# Autodesk Inventor assembly: PruebaIntegracion
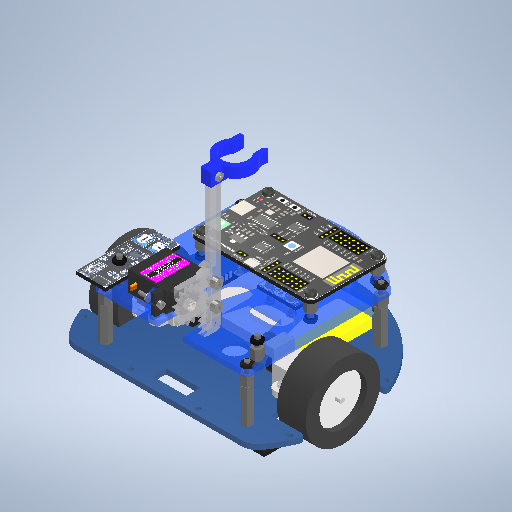
[picture p0: Inventor's stored thumbnail of the model, 512x512]
Saved by Autodesk Inventor 2025.2 (Build 292293000, 293)
## iProperties
Created: 2025-04-23
Part Number: PruebaIntegracion
Document SubType Name: Assembly
Designer: cdavi
Author: cdavi
## Documents named in this file (34)
- D:\Documentos\GIRoM\Atta-Bot-STEM\Chasis\Rediseño_Diego&Carlos\PruebaIntegracion.iam
- D:\Documentos\GIRoM\Atta-Bot-STEM\Chasis\Rediseño_Diego&Carlos\base_chasis_v5\base_chasis_v4-dimsAjustadas.ipt
- D:\Documentos\GIRoM\Atta-Bot-STEM\Chasis\Rediseño_Diego&Carlos\base_chasis_v5.ipt
- D:\Documentos\GIRoM\Atta-Bot-STEM\Chasis\Rediseño_Diego&Carlos\base_nivel2.ipt
- D:\Documentos\GIRoM\Atta-Bot-STEM\Chasis\Rediseño_Diego&Carlos\spacers\hexagonal_spacer_MF_M3_H20_HEX5.5_FTD6_MTL6.ipt
- D:\Documentos\GIRoM\Atta-Bot-STEM\Chasis\Rediseño_Diego&Carlos\spacers\hexagonal_spacer_MF_M3_H06_HEX5.5_FTD3_MTL6.ipt
- D:\Documentos\GIRoM\Atta-Bot-STEM\Chasis\Rediseño_Diego&Carlos\base_powerboost.ipt
- D:\Documentos\GIRoM\Atta-Bot-STEM\Chasis\Rediseño_Diego&Carlos\ideaboard.ipt
- D:\Documentos\Inventor\Content Center Files\R2025\en-US\ISO 4032(2)\ISO 4032 - M3 - ISO.ipt
- D:\Documentos\GIRoM\Atta-Bot-STEM\Chasis\Rediseño_Diego&Carlos\sensorFrontal.ipt
- D:\Documentos\Inventor\Content Center Files\R2025\en-US\ISO 7045  Z\ISO 7045 - M3 x 6_ - 4.8 - Z - ISO.ipt
- D:\Documentos\GIRoM\Atta-Bot-STEM\Chasis\Rediseño_Diego&Carlos\sensorInferior.ipt
- D:\Documentos\GIRoM\Atta-Bot-STEM\Chasis\Rediseño_Diego&Carlos\powerboost.ipt
- D:\Documentos\Inventor\Content Center Files\R2025\en-US\ISO 4762(2)\ISO 4762 - M2 x 8ISO.ipt
- D:\Documentos\Inventor\Content Center Files\R2025\en-US\ISO 4032(2)\ISO 4032 - M2 - ISO.ipt
- D:\Documentos\GIRoM\Atta-Bot-STEM\Chasis\Rediseño_Diego&Carlos\bateria.ipt
- D:\Documentos\GIRoM\Atta-Bot-STEM\Chasis\Rediseño_Diego&Carlos\soporteMotor.ipt
- D:\Documentos\GIRoM\Atta-Bot-STEM\Chasis\Rediseño_Diego&Carlos\motor.ipt
- D:\Documentos\GIRoM\Atta-Bot-STEM\Chasis\Rediseño_Diego&Carlos\llanta.ipt
- D:\Documentos\GIRoM\Atta-Bot-STEM\Chasis\Rediseño_Diego&Carlos\ball_caster.ipt
- D:\Documentos\Inventor\Content Center Files\R2025\en-US\ISO 4762(2)\ISO 4762 - M2 x 12ISO.ipt
- D:\Documentos\GIRoM\Atta-Bot-STEM\Chasis\Rediseño_Diego&Carlos\switch.ipt
- D:\Documentos\GIRoM\Atta-Bot-STEM\Chasis\Rediseño_Diego&Carlos\Tower Pro MG90S Micro servo.ipt
- D:\Documentos\GIRoM\Atta-Bot-STEM\Chasis\Rediseño_Diego&Carlos\EngraneMod_v2.ipt
- D:\Documentos\GIRoM\Atta-Bot-STEM\Chasis\Rediseño_Diego&Carlos\sujetador_cremallera.ipt
- D:\Documentos\GIRoM\Atta-Bot-STEM\Chasis\Rediseño_Diego&Carlos\cremallera_v2\cremallera-01.ipt
- D:\Documentos\GIRoM\Atta-Bot-STEM\Chasis\Rediseño_Diego&Carlos\cremallera_v2.ipt
- D:\Documentos\GIRoM\Atta-Bot-STEM\Chasis\Rediseño_Diego&Carlos\sujetador_marcador_v2.ipt
- D:\Documentos\Inventor\Content Center Files\R2025\en-US\ISO 7045  Z\ISO 7045 - M1,6 x 6_ - 4.8 - Z - ISO.ipt
- D:\Documentos\Inventor\Content Center Files\R2025\en-US\ISO 4762(2)\ISO 4762 - M3 x 8ISO.ipt
- D:\Documentos\GIRoM\Atta-Bot-STEM\Chasis\Rediseño_Diego&Carlos\SoporteServo.ipt
- D:\Documentos\2025\Semestre 1\Robótica\Proyecto\carcasa_v2.4.ipt
- D:\Documentos\GIRoM\Atta-Bot-STEM\Chasis\Rediseño_Diego&Carlos\spacers\hexagonal_spacer_MF_M3_H08_HEX5_FTD4_MTL8.ipt
- D:\Documentos\Inventor\Content Center Files\R2025\en-US\ISO 4762(2)\ISO 4762 - M3 x 12ISO.ipt
## Components (110 placed, 31 different names)
1. carcasa_v2.4:1 — Mate:183, Mate:184, Mate:185
2. hexagonal_spacer_MF_M3_H20_HEX5.5_FTD6_MTL6:1 — Mate:3, Mate:4
3. hexagonal_spacer_MF_M3_H20_HEX5.5_FTD6_MTL6:2 — Mate:5, Mate:6
4. hexagonal_spacer_MF_M3_H20_HEX5.5_FTD6_MTL6:3 — Mate:7, Mate:8
5. hexagonal_spacer_MF_M3_H20_HEX5.5_FTD6_MTL6:4 — Mate:9, Mate:10
6. hexagonal_spacer_MF_M3_H06_HEX5.5_FTD3_MTL6:7
7. hexagonal_spacer_MF_M3_H06_HEX5.5_FTD3_MTL6:8
8. hexagonal_spacer_MF_M3_H06_HEX5.5_FTD3_MTL6:9
9. hexagonal_spacer_MF_M3_H06_HEX5.5_FTD3_MTL6:10
10. hexagonal_spacer_MF_M3_H08_HEX5_FTD4_MTL8:2
11. hexagonal_spacer_MF_M3_H08_HEX5_FTD4_MTL8:1
12. hexagonal_spacer_MF_M3_H08_HEX5_FTD4_MTL8:3
13. hexagonal_spacer_MF_M3_H08_HEX5_FTD4_MTL8:4
14. hexagonal_spacer_MF_M3_H06_HEX5.5_FTD3_MTL6:2 — Mate:44, Mate:45
15. hexagonal_spacer_MF_M3_H06_HEX5.5_FTD3_MTL6:3 — Mate:48, Mate:49
16. hexagonal_spacer_MF_M3_H06_HEX5.5_FTD3_MTL6:1 — Mate:42, Mate:43, Mate:50, Mate:51
17. hexagonal_spacer_MF_M3_H06_HEX5.5_FTD3_MTL6:4 — Mate:46, Mate:47, Mate:52
18. hexagonal_spacer_MF_M3_H06_HEX5.5_FTD3_MTL6:5 — Mate:53, Mate:54, Mate:68, Mate:69, Mate:70
19. hexagonal_spacer_MF_M3_H06_HEX5.5_FTD3_MTL6:6 — Mate:55, Mate:56, Mate:66, Mate:67, Mate:73
20. ISO 4032 M3:17 — Mate:199, Mate:83
21. ISO 4032 M3:18 — Mate:201, Mate:85
22. ISO 7045 Z M3 x 6 - 4.8 - Z:11 — Insert:14
23. ISO 7045 Z M3 x 6 - 4.8 - Z:12 — Insert:15
24. ISO 4032 M3:13 — Insert:16
25. ISO 4032 M3:14 — Insert:17
26. ISO 4032 M3:15 — Insert:18
27. ISO 4032 M3:16 — Insert:19
28. ISO 4032 M3:7 — Insert:5
29. ISO 4032 M3:8 — Insert:6
30. ISO 4032 M3:9 — Insert:7
31. ISO 4032 M3:10 — Insert:8
32. ISO 7045 Z M3 x 6 - 4.8 - Z:10 — Insert:9
33. ISO 7045 Z M3 x 6 - 4.8 - Z:9 — Insert:10
34. ISO 4762 M3 x 12:1 — Insert:114
35. ISO 4762 M3 x 12:2 — Mate:115, Mate:116
36. ISO 7045 Z M3 x 6 - 4.8 - Z:5 — Mate:89, Mate:90
37. ISO 7045 Z M3 x 6 - 4.8 - Z:6 — Mate:91, Mate:92
38. ISO 7045 Z M3 x 6 - 4.8 - Z:7 — Mate:93, Mate:94
39. ISO 7045 Z M3 x 6 - 4.8 - Z:8 — Mate:95, Mate:96
40. ISO 4032 M3:1 — Mate:58
41. ISO 4032 M3:2 — Mate:60
42. ISO 4032 M3:3 — Mate:63
43. ISO 4032 M3:4 — Mate:64
44. ISO 4032 M3:5 — Mate:70, Mate:71
45. ISO 4032 M3:6 — Mate:72, Mate:73
46. ISO 7045 Z M3 x 6 - 4.8 - Z:1 — Mate:74, Mate:75
47. ISO 7045 Z M3 x 6 - 4.8 - Z:2 — Mate:76, Mate:77
48. ISO 7045 Z M3 x 6 - 4.8 - Z:3 — Mate:78, Mate:79
49. ISO 7045 Z M3 x 6 - 4.8 - Z:4 — Mate:80, Mate:81
50. ISO 4032 M2:14 — Mate:189, Mate:190
51. ISO 4032 M2:15 — Mate:191, Mate:192
52. ISO 4032 M2:16 — Mate:193, Mate:194, Mate:197
53. ISO 4032 M2:17 — Mate:195, Mate:196
54. ISO 4762 M2 x 8:4 — Mate:148, Mate:149, Mate:154
55. ISO 4762 M2 x 8:5 — Mate:150, Mate:151, Mate:152
56. ISO 4032 M2:6 — Mate:152, Mate:153
57. ISO 4032 M2:7 — Mate:154, Mate:155
58. ISO 4032 M2:8 — Mate:160, Mate:161
59. ISO 4032 M2:9 — Mate:162, Mate:163
60. ISO 4032 M2:10 — Mate:164, Mate:165
61. ISO 4032 M2:11 — Mate:166, Mate:167
62. ISO 4762 M2 x 8:9 — Mate:160
63. ISO 4762 M2 x 8:6 — Mate:162
64. ISO 4762 M2 x 8:7 — Mate:166
65. ISO 4762 M2 x 8:8 — Mate:164
66. ISO 4762 M2 x 8:1 — Mate:97, Mate:98, Mate:110, Mate:191
67. ISO 4762 M2 x 8:2 — Mate:99, Mate:100, Mate:112, Mate:189
68. ISO 4762 M2 x 12:2 — Mate:101, Mate:102, Mate:105, Mate:195
69. ISO 4762 M2 x 12:3 — Mate:103, Mate:104, Mate:108, Mate:193
70. ISO 4032 M2:1 — Mate:105, Mate:106
71. ISO 4032 M2:2 — Mate:107, Mate:108
72. ISO 4032 M2:3 — Mate:109, Mate:110
73. ISO 4032 M2:4 — Mate:111, Mate:112
74. ISO 7045 Z M1,6 x 6 - 4.8 - Z:2 — Mate:156, Mate:157
75. ISO 7045 Z M1,6 x 6 - 4.8 - Z:1 — Mate:158, Mate:159
76. bateria:1 — Mate:119, Mate:120
77. soporteMotor:1 — Mate:117, Mate:118, Angle:8, Mate:124, Tangent:2
78. soporteMotor:2 — Mate:119, Mate:122, Tangent:1, Mate:181, Angle:12, Mate:182
79. motor:1 — Mate:122, Tangent:1, Mate:123, Mate:126, Flush:5, Mate:127
80. motor:2 — Mate:124, Tangent:2, Mate:125, Mate:128, Mate:129, Flush:6
81. llanta:1 — Mate:126, Flush:5, Mate:127
82. llanta:2 — Mate:128, Mate:129, Flush:6
83. ball_caster:1 — Tangent:3, Tangent:7, Mate:130, Mate:156, Mate:158
84. switch:1 — Mate:131, Mate:132, Mate:133, Mate:148, Mate:149, Mate:150, Mate:151
85. sensorInferior:2 — Angle:7, Mate:85, Insert:114, Mate:82
86. sensorInferior:1 — Angle:6, Mate:83, Mate:115, Mate:116, Mate:84
87. powerboost:1 — Mate:86, Mate:87, Mate:88, Mate:97, Mate:98, Mate:99, Mate:100, Mate:101, Mate:102, Mate:103, Mate:104, Mate:197
88. base_chasis_v4-dimsAjustadas:1 — Mate:1, Flush:8, Flush:4, Mate:3, Mate:4, Mate:5, Mate:6, Mate:7, Mate:8, Mate:9, Mate:10, Mate:82, Angle:6, Mate:84, Angle:7, Mate:117, Mate:118, Angle:8, Mate:120, Mate:123, Mate:125, Tangent:3, Tangent:7, Mate:130, Mate:131, Mate:132, Mate:133, Mate:153, Mate:155, Mate:157, Mate:159, Mate:161, Mate:163, Mate:165, Mate:167, Insert:5, Insert:6, Insert:7, Insert:8, Insert:9, Insert:10, Mate:181, Angle:12, Mate:182, Mate:183, Mate:184, Mate:185, Mate:199, Mate:201
89. base_powerboost:1 — Mate:86, Mate:87, Mate:88, Mate:89, Mate:90, Mate:91, Mate:92, Mate:93, Mate:94, Mate:95, Mate:96, Mate:106, Mate:107, Mate:109, Mate:111, Mate:190, Mate:192, Mate:194, Mate:196
90. SoporteServo:2 — Mate:186, Mate:187, Mate:188, Mate:209
91. base_nivel2:1 — Mate:42, Mate:43, Mate:44, Mate:45, Mate:46, Mate:47, Mate:48, Mate:49, Mate:53, Mate:54, Mate:55, Mate:56, Mate:58, Mate:60, Mate:63, Mate:64, Angle:4, Angle:5, Angle:9, Insert:14, Insert:15, Insert:16, Insert:17, Insert:18, Insert:19, Flush:7, Mate:186, Mate:187
92. SoporteServo:1 — Mate:208
93. ideaboard:1 — Mate:50, Mate:51, Mate:52, Mate:74, Mate:75, Mate:76, Mate:77, Mate:78, Mate:79, Mate:80, Mate:81
94. sensorFrontal:1 — Mate:66, Mate:67, Angle:4, Mate:72
95. sensorFrontal:2 — Mate:68, Mate:69, Angle:5, Mate:71
96. ISO 4032 M2:13 — Mate:179, Mate:208
97. ISO 4032 M2:12 — Mate:177, Mate:209
98. ISO 4762 M2 x 12:5 — Insert:13, Mate:177
99. ISO 4762 M3 x 8:1 — Mate:202, Mate:203, Mate:206
100. ISO 4762 M3 x 8:2 — Mate:204, Mate:205, Mate:207
101. ISO 4032 M3:11 — Mate:169, Mate:206
102. ISO 4032 M3:12 — Mate:171, Mate:207
103. ISO 4762 M2 x 12:4 — Mate:172, Mate:173, Mate:179
104. Tower Pro MG90S Micro servo:1 — Angle:9, Mate:136, Mate:138, Angle:10, Mate:143, Mate:172, Mate:173, Insert:13, Flush:7, Mate:188
105. EngraneMod_v2:1 — Mate:136, Mate:139, Mate:143
106. sujetador_cremallera:1 — Mate:138, Angle:10, Mate:139, Tangent:5, Tangent:6, Mate:140, Mate:203, Mate:205, Mate:169, Mate:171
107. cremallera-01:1 — Tangent:5, Tangent:6, Mate:140, Mate:141, Angle:11, Mate:142, Mate:202, Mate:204
108. sujetador_marcador_v2:1 — Mate:141, Angle:11, Mate:142, Mate:144, Mate:145, Mate:147
109. ISO 4762 M2 x 8:3 — Mate:144, Mate:145, Mate:146
110. ISO 4032 M2:5 — Mate:146, Mate:147
## Relationships (226: Mate 188, Insert 18, Angle 9, Tangent 6, Flush 5)
- Mate:1: base_chasis_v4-dimsAjustadas:1
- Flush:8: base_chasis_v4-dimsAjustadas:1
- Flush:4: base_chasis_v4-dimsAjustadas:1
- Mate:3: hexagonal_spacer_MF_M3_H20_HEX5.5_FTD6_MTL6:1 ↔ base_chasis_v4-dimsAjustadas:1
- Mate:4: hexagonal_spacer_MF_M3_H20_HEX5.5_FTD6_MTL6:1 ↔ base_chasis_v4-dimsAjustadas:1
- Mate:5: hexagonal_spacer_MF_M3_H20_HEX5.5_FTD6_MTL6:2 ↔ base_chasis_v4-dimsAjustadas:1
- Mate:6: hexagonal_spacer_MF_M3_H20_HEX5.5_FTD6_MTL6:2 ↔ base_chasis_v4-dimsAjustadas:1
- Mate:7: hexagonal_spacer_MF_M3_H20_HEX5.5_FTD6_MTL6:3 ↔ base_chasis_v4-dimsAjustadas:1
- Mate:8: hexagonal_spacer_MF_M3_H20_HEX5.5_FTD6_MTL6:3 ↔ base_chasis_v4-dimsAjustadas:1
- Mate:9: hexagonal_spacer_MF_M3_H20_HEX5.5_FTD6_MTL6:4 ↔ base_chasis_v4-dimsAjustadas:1
- Mate:10: hexagonal_spacer_MF_M3_H20_HEX5.5_FTD6_MTL6:4 ↔ base_chasis_v4-dimsAjustadas:1
- [Mate]: hexagonal_spacer_MF_M3_H20_HEX5.5_FTD6_MTL6:2 ↔ hexagonal_spacer_MF_M3_H06_HEX5.5_FTD3_MTL6:7
- [Mate]: hexagonal_spacer_MF_M3_H20_HEX5.5_FTD6_MTL6:2 ↔ hexagonal_spacer_MF_M3_H06_HEX5.5_FTD3_MTL6:7
- [Mate]: hexagonal_spacer_MF_M3_H20_HEX5.5_FTD6_MTL6:1 ↔ hexagonal_spacer_MF_M3_H06_HEX5.5_FTD3_MTL6:10
- [Mate]: hexagonal_spacer_MF_M3_H20_HEX5.5_FTD6_MTL6:1 ↔ hexagonal_spacer_MF_M3_H06_HEX5.5_FTD3_MTL6:10
- [Mate]: hexagonal_spacer_MF_M3_H20_HEX5.5_FTD6_MTL6:4 ↔ hexagonal_spacer_MF_M3_H06_HEX5.5_FTD3_MTL6:9
- [Mate]: hexagonal_spacer_MF_M3_H20_HEX5.5_FTD6_MTL6:4 ↔ hexagonal_spacer_MF_M3_H06_HEX5.5_FTD3_MTL6:9
- [Mate]: hexagonal_spacer_MF_M3_H20_HEX5.5_FTD6_MTL6:3 ↔ hexagonal_spacer_MF_M3_H06_HEX5.5_FTD3_MTL6:8
- [Mate]: hexagonal_spacer_MF_M3_H20_HEX5.5_FTD6_MTL6:3 ↔ hexagonal_spacer_MF_M3_H06_HEX5.5_FTD3_MTL6:8
- [Mate]: hexagonal_spacer_MF_M3_H06_HEX5.5_FTD3_MTL6:7 ↔ base_nivel2:1
- [Mate]: hexagonal_spacer_MF_M3_H06_HEX5.5_FTD3_MTL6:9 ↔ base_nivel2:1
- [Mate]: hexagonal_spacer_MF_M3_H06_HEX5.5_FTD3_MTL6:7 ↔ base_nivel2:1
- [Mate]: hexagonal_spacer_MF_M3_H08_HEX5_FTD4_MTL8:2 ↔ base_chasis_v4-dimsAjustadas:1
- [Mate]: hexagonal_spacer_MF_M3_H08_HEX5_FTD4_MTL8:2 ↔ base_chasis_v4-dimsAjustadas:1
- [Mate]: hexagonal_spacer_MF_M3_H08_HEX5_FTD4_MTL8:1 ↔ base_chasis_v4-dimsAjustadas:1
- [Mate]: hexagonal_spacer_MF_M3_H08_HEX5_FTD4_MTL8:1 ↔ base_chasis_v4-dimsAjustadas:1
- [Mate]: hexagonal_spacer_MF_M3_H08_HEX5_FTD4_MTL8:3 ↔ base_chasis_v4-dimsAjustadas:1
- [Mate]: hexagonal_spacer_MF_M3_H08_HEX5_FTD4_MTL8:3 ↔ base_chasis_v4-dimsAjustadas:1
- [Mate]: hexagonal_spacer_MF_M3_H08_HEX5_FTD4_MTL8:4 ↔ base_chasis_v4-dimsAjustadas:1
- [Mate]: hexagonal_spacer_MF_M3_H08_HEX5_FTD4_MTL8:4 ↔ base_chasis_v4-dimsAjustadas:1
- [Mate]: hexagonal_spacer_MF_M3_H08_HEX5_FTD4_MTL8:3 ↔ base_powerboost:1
- [Mate]: hexagonal_spacer_MF_M3_H08_HEX5_FTD4_MTL8:2 ↔ base_powerboost:1
- [Mate]: hexagonal_spacer_MF_M3_H08_HEX5_FTD4_MTL8:2 ↔ base_powerboost:1
- [Mate]: base_nivel2:1 ↔ SoporteServo:1
- [Mate]: base_nivel2:1 ↔ SoporteServo:1
- [Mate]: base_nivel2:1 ↔ SoporteServo:1
- Mate:42: hexagonal_spacer_MF_M3_H06_HEX5.5_FTD3_MTL6:1 ↔ base_nivel2:1
- Mate:43: hexagonal_spacer_MF_M3_H06_HEX5.5_FTD3_MTL6:1 ↔ base_nivel2:1
- Mate:44: hexagonal_spacer_MF_M3_H06_HEX5.5_FTD3_MTL6:2 ↔ base_nivel2:1
- Mate:45: hexagonal_spacer_MF_M3_H06_HEX5.5_FTD3_MTL6:2 ↔ base_nivel2:1
- Mate:46: hexagonal_spacer_MF_M3_H06_HEX5.5_FTD3_MTL6:4 ↔ base_nivel2:1
- Mate:47: hexagonal_spacer_MF_M3_H06_HEX5.5_FTD3_MTL6:4 ↔ base_nivel2:1
- Mate:48: hexagonal_spacer_MF_M3_H06_HEX5.5_FTD3_MTL6:3 ↔ base_nivel2:1
- Mate:49: hexagonal_spacer_MF_M3_H06_HEX5.5_FTD3_MTL6:3 ↔ base_nivel2:1
- Mate:50: hexagonal_spacer_MF_M3_H06_HEX5.5_FTD3_MTL6:1 ↔ ideaboard:1
- Mate:51: hexagonal_spacer_MF_M3_H06_HEX5.5_FTD3_MTL6:1 ↔ ideaboard:1
- Mate:52: hexagonal_spacer_MF_M3_H06_HEX5.5_FTD3_MTL6:4 ↔ ideaboard:1
- Mate:53: hexagonal_spacer_MF_M3_H06_HEX5.5_FTD3_MTL6:5 ↔ base_nivel2:1
- Mate:54: hexagonal_spacer_MF_M3_H06_HEX5.5_FTD3_MTL6:5 ↔ base_nivel2:1
- Mate:55: hexagonal_spacer_MF_M3_H06_HEX5.5_FTD3_MTL6:6 ↔ base_nivel2:1
- Mate:56: hexagonal_spacer_MF_M3_H06_HEX5.5_FTD3_MTL6:6 ↔ base_nivel2:1
- [Mate]: hexagonal_spacer_MF_M3_H06_HEX5.5_FTD3_MTL6:8 ↔ ISO 4032 M3:1
- Mate:58: ISO 4032 M3:1 ↔ base_nivel2:1
- Mate:60: ISO 4032 M3:2 ↔ base_nivel2:1
- [Mate]: hexagonal_spacer_MF_M3_H06_HEX5.5_FTD3_MTL6:7 ↔ ISO 4032 M3:2
- [Mate]: hexagonal_spacer_MF_M3_H06_HEX5.5_FTD3_MTL6:10 ↔ ISO 4032 M3:3
- Mate:63: ISO 4032 M3:3 ↔ base_nivel2:1
- Mate:64: ISO 4032 M3:4 ↔ base_nivel2:1
- [Mate]: hexagonal_spacer_MF_M3_H06_HEX5.5_FTD3_MTL6:9 ↔ ISO 4032 M3:4
- Mate:66: hexagonal_spacer_MF_M3_H06_HEX5.5_FTD3_MTL6:6 ↔ sensorFrontal:1
- Mate:67: hexagonal_spacer_MF_M3_H06_HEX5.5_FTD3_MTL6:6 ↔ sensorFrontal:1
- Angle:4 (180 deg): base_nivel2:1 ↔ sensorFrontal:1
- Mate:68: hexagonal_spacer_MF_M3_H06_HEX5.5_FTD3_MTL6:5 ↔ sensorFrontal:2
- Mate:69: hexagonal_spacer_MF_M3_H06_HEX5.5_FTD3_MTL6:5 ↔ sensorFrontal:2
- Angle:5 (0 deg): base_nivel2:1 ↔ sensorFrontal:2
- Mate:70: hexagonal_spacer_MF_M3_H06_HEX5.5_FTD3_MTL6:5 ↔ ISO 4032 M3:5
- Mate:71: ISO 4032 M3:5 ↔ sensorFrontal:2
- Mate:72: ISO 4032 M3:6 ↔ sensorFrontal:1
- Mate:73: hexagonal_spacer_MF_M3_H06_HEX5.5_FTD3_MTL6:6 ↔ ISO 4032 M3:6
- Mate:74: ISO 7045 Z M3 x 6 - 4.8 - Z:1 ↔ ideaboard:1
- Mate:75: ISO 7045 Z M3 x 6 - 4.8 - Z:1 ↔ ideaboard:1
- Mate:76: ISO 7045 Z M3 x 6 - 4.8 - Z:2 ↔ ideaboard:1
- Mate:77: ISO 7045 Z M3 x 6 - 4.8 - Z:2 ↔ ideaboard:1
- Mate:78: ISO 7045 Z M3 x 6 - 4.8 - Z:3 ↔ ideaboard:1
- Mate:79: ISO 7045 Z M3 x 6 - 4.8 - Z:3 ↔ ideaboard:1
- Mate:80: ISO 7045 Z M3 x 6 - 4.8 - Z:4 ↔ ideaboard:1
- Mate:81: ISO 7045 Z M3 x 6 - 4.8 - Z:4 ↔ ideaboard:1
- Mate:82: sensorInferior:2 ↔ base_chasis_v4-dimsAjustadas:1
- Angle:6 (0 deg): sensorInferior:1 ↔ base_chasis_v4-dimsAjustadas:1
- Mate:83: ISO 4032 M3:17 ↔ sensorInferior:1
- Mate:84: sensorInferior:1 ↔ base_chasis_v4-dimsAjustadas:1
- Angle:7 (0 deg): sensorInferior:2 ↔ base_chasis_v4-dimsAjustadas:1
- Mate:85: ISO 4032 M3:18 ↔ sensorInferior:2
- Mate:86: powerboost:1 ↔ base_powerboost:1
- Mate:87: powerboost:1 ↔ base_powerboost:1
- Mate:88 (1 mm): powerboost:1 ↔ base_powerboost:1
- Mate:89: ISO 7045 Z M3 x 6 - 4.8 - Z:5 ↔ base_powerboost:1
- Mate:90: ISO 7045 Z M3 x 6 - 4.8 - Z:5 ↔ base_powerboost:1
- Mate:91: ISO 7045 Z M3 x 6 - 4.8 - Z:6 ↔ base_powerboost:1
- Mate:92: ISO 7045 Z M3 x 6 - 4.8 - Z:6 ↔ base_powerboost:1
- Mate:93: ISO 7045 Z M3 x 6 - 4.8 - Z:7 ↔ base_powerboost:1
- Mate:94: ISO 7045 Z M3 x 6 - 4.8 - Z:7 ↔ base_powerboost:1
- Mate:95: ISO 7045 Z M3 x 6 - 4.8 - Z:8 ↔ base_powerboost:1
- Mate:96: ISO 7045 Z M3 x 6 - 4.8 - Z:8 ↔ base_powerboost:1
- Mate:97: ISO 4762 M2 x 8:1 ↔ powerboost:1
- Mate:98: ISO 4762 M2 x 8:1 ↔ powerboost:1
- Mate:99: ISO 4762 M2 x 8:2 ↔ powerboost:1
- Mate:100: ISO 4762 M2 x 8:2 ↔ powerboost:1
- Mate:101: ISO 4762 M2 x 12:2 ↔ powerboost:1
- Mate:102: ISO 4762 M2 x 12:2 ↔ powerboost:1
- Mate:103: ISO 4762 M2 x 12:3 ↔ powerboost:1
- Mate:104: ISO 4762 M2 x 12:3 ↔ powerboost:1
- Mate:105: ISO 4762 M2 x 12:2 ↔ ISO 4032 M2:1
- Mate:106: ISO 4032 M2:1 ↔ base_powerboost:1
- Mate:107: ISO 4032 M2:2 ↔ base_powerboost:1
- Mate:108: ISO 4762 M2 x 12:3 ↔ ISO 4032 M2:2
- Mate:109: ISO 4032 M2:3 ↔ base_powerboost:1
- Mate:110: ISO 4762 M2 x 8:1 ↔ ISO 4032 M2:3
- Mate:111: ISO 4032 M2:4 ↔ base_powerboost:1
- Mate:112: ISO 4762 M2 x 8:2 ↔ ISO 4032 M2:4
- Insert:114: ISO 4762 M3 x 12:1 ↔ sensorInferior:2
- Mate:115: ISO 4762 M3 x 12:2 ↔ sensorInferior:1
- Mate:116: ISO 4762 M3 x 12:2 ↔ sensorInferior:1
- Mate:117: soporteMotor:1 ↔ base_chasis_v4-dimsAjustadas:1
- Mate:118: soporteMotor:1 ↔ base_chasis_v4-dimsAjustadas:1
- Angle:8 (0 deg): soporteMotor:1 ↔ base_chasis_v4-dimsAjustadas:1
- Mate:119: bateria:1 ↔ soporteMotor:2
- Mate:120: bateria:1 ↔ base_chasis_v4-dimsAjustadas:1
- [Mate] (1 mm): hexagonal_spacer_MF_M3_H08_HEX5_FTD4_MTL8:1 ↔ bateria:1
- Mate:122: soporteMotor:2 ↔ motor:1
- Tangent:1: soporteMotor:2 ↔ motor:1
- Mate:123: motor:1 ↔ base_chasis_v4-dimsAjustadas:1
- Mate:124: soporteMotor:1 ↔ motor:2
- Tangent:2: soporteMotor:1 ↔ motor:2
- Mate:125: motor:2 ↔ base_chasis_v4-dimsAjustadas:1
- Mate:126: motor:1 ↔ llanta:1
- Flush:5 (-3 mm): motor:1 ↔ llanta:1
- Mate:127: motor:1 ↔ llanta:1
- Mate:128: motor:2 ↔ llanta:2
- Mate:129: motor:2 ↔ llanta:2
- Flush:6 (-3 mm): motor:2 ↔ llanta:2
- Tangent:3: ball_caster:1 ↔ base_chasis_v4-dimsAjustadas:1
- Tangent:7: ball_caster:1 ↔ base_chasis_v4-dimsAjustadas:1
- Mate:130: ball_caster:1 ↔ base_chasis_v4-dimsAjustadas:1
- Mate:131: switch:1 ↔ base_chasis_v4-dimsAjustadas:1
- Mate:132: switch:1 ↔ base_chasis_v4-dimsAjustadas:1
- Mate:133 (0.2 mm): switch:1 ↔ base_chasis_v4-dimsAjustadas:1
- [Mate]: SoporteServo:1 ↔ Tower Pro MG90S Micro servo:1
- Angle:9 (180 deg): base_nivel2:1 ↔ Tower Pro MG90S Micro servo:1
- Mate:136: Tower Pro MG90S Micro servo:1 ↔ EngraneMod_v2:1
- Mate:138: Tower Pro MG90S Micro servo:1 ↔ sujetador_cremallera:1
- Angle:10 (0 deg): Tower Pro MG90S Micro servo:1 ↔ sujetador_cremallera:1
- Mate:139: EngraneMod_v2:1 ↔ sujetador_cremallera:1
- Tangent:5: sujetador_cremallera:1 ↔ cremallera-01:1
- Tangent:6: sujetador_cremallera:1 ↔ cremallera-01:1
- Mate:140: sujetador_cremallera:1 ↔ cremallera-01:1
- Mate:141: cremallera-01:1 ↔ sujetador_marcador_v2:1
- Angle:11 (0 deg): cremallera-01:1 ↔ sujetador_marcador_v2:1
- Mate:142: cremallera-01:1 ↔ sujetador_marcador_v2:1
- Mate:143: Tower Pro MG90S Micro servo:1 ↔ EngraneMod_v2:1
- Mate:144: sujetador_marcador_v2:1 ↔ ISO 4762 M2 x 8:3
- Mate:145: sujetador_marcador_v2:1 ↔ ISO 4762 M2 x 8:3
- Mate:146: ISO 4762 M2 x 8:3 ↔ ISO 4032 M2:5
- Mate:147: sujetador_marcador_v2:1 ↔ ISO 4032 M2:5
- Mate:148: ISO 4762 M2 x 8:4 ↔ switch:1
- Mate:149: ISO 4762 M2 x 8:4 ↔ switch:1
- Mate:150: ISO 4762 M2 x 8:5 ↔ switch:1
- Mate:151: ISO 4762 M2 x 8:5 ↔ switch:1
- Mate:152: ISO 4762 M2 x 8:5 ↔ ISO 4032 M2:6
- Mate:153: ISO 4032 M2:6 ↔ base_chasis_v4-dimsAjustadas:1
- Mate:154: ISO 4762 M2 x 8:4 ↔ ISO 4032 M2:7
- Mate:155: ISO 4032 M2:7 ↔ base_chasis_v4-dimsAjustadas:1
- Mate:156: ISO 7045 Z M1,6 x 6 - 4.8 - Z:2 ↔ ball_caster:1
- Mate:157: ISO 7045 Z M1,6 x 6 - 4.8 - Z:2 ↔ base_chasis_v4-dimsAjustadas:1
- Mate:158: ISO 7045 Z M1,6 x 6 - 4.8 - Z:1 ↔ ball_caster:1
- Mate:159: ISO 7045 Z M1,6 x 6 - 4.8 - Z:1 ↔ base_chasis_v4-dimsAjustadas:1
- [Insert]: ISO 4762 M2 x 8:9 ↔ soporteMotor:2
- [Insert]: ISO 4762 M2 x 8:6 ↔ soporteMotor:2
- [Insert]: ISO 4762 M2 x 8:7 ↔ soporteMotor:1
- [Insert]: ISO 4762 M2 x 8:8 ↔ soporteMotor:1
- Mate:160: ISO 4032 M2:8 ↔ ISO 4762 M2 x 8:9
- Mate:161: ISO 4032 M2:8 ↔ base_chasis_v4-dimsAjustadas:1
- Mate:162: ISO 4032 M2:9 ↔ ISO 4762 M2 x 8:6
- Mate:163: ISO 4032 M2:9 ↔ base_chasis_v4-dimsAjustadas:1
- Mate:164: ISO 4032 M2:10 ↔ ISO 4762 M2 x 8:8
- Mate:165: ISO 4032 M2:10 ↔ base_chasis_v4-dimsAjustadas:1
- Mate:166: ISO 4032 M2:11 ↔ ISO 4762 M2 x 8:7
- Mate:167: ISO 4032 M2:11 ↔ base_chasis_v4-dimsAjustadas:1
- Insert:5: ISO 4032 M3:7 ↔ base_chasis_v4-dimsAjustadas:1
- Insert:6: ISO 4032 M3:8 ↔ base_chasis_v4-dimsAjustadas:1
- Insert:7: ISO 4032 M3:9 ↔ base_chasis_v4-dimsAjustadas:1
- Insert:8: ISO 4032 M3:10 ↔ base_chasis_v4-dimsAjustadas:1
- Insert:9: ISO 7045 Z M3 x 6 - 4.8 - Z:10 ↔ base_chasis_v4-dimsAjustadas:1
- Insert:10: ISO 7045 Z M3 x 6 - 4.8 - Z:9 ↔ base_chasis_v4-dimsAjustadas:1
- Mate:169: ISO 4032 M3:11 ↔ sujetador_cremallera:1
- Mate:171: ISO 4032 M3:12 ↔ sujetador_cremallera:1
- Mate:172: ISO 4762 M2 x 12:4 ↔ Tower Pro MG90S Micro servo:1
- Mate:173: ISO 4762 M2 x 12:4 ↔ Tower Pro MG90S Micro servo:1
- Insert:13: ISO 4762 M2 x 12:5 ↔ Tower Pro MG90S Micro servo:1
- Mate:177: ISO 4032 M2:12 ↔ ISO 4762 M2 x 12:5
- Mate:179: ISO 4032 M2:13 ↔ ISO 4762 M2 x 12:4
- Insert:14: ISO 7045 Z M3 x 6 - 4.8 - Z:11 ↔ base_nivel2:1
- Insert:15: ISO 7045 Z M3 x 6 - 4.8 - Z:12 ↔ base_nivel2:1
- Insert:16: ISO 4032 M3:13 ↔ base_nivel2:1
- Insert:17: ISO 4032 M3:14 ↔ base_nivel2:1
- Insert:18: ISO 4032 M3:15 ↔ base_nivel2:1
- Insert:19: ISO 4032 M3:16 ↔ base_nivel2:1
- Flush:7: base_nivel2:1 ↔ Tower Pro MG90S Micro servo:1
- Mate:181: soporteMotor:2 ↔ base_chasis_v4-dimsAjustadas:1
- Angle:12 (0 deg): soporteMotor:2 ↔ base_chasis_v4-dimsAjustadas:1
- Mate:182: soporteMotor:2 ↔ base_chasis_v4-dimsAjustadas:1
- Mate:183: carcasa_v2.4:1 ↔ base_chasis_v4-dimsAjustadas:1
- Mate:184: carcasa_v2.4:1 ↔ base_chasis_v4-dimsAjustadas:1
- Mate:185 (0.002 mm): carcasa_v2.4:1 ↔ base_chasis_v4-dimsAjustadas:1
- Mate:186: SoporteServo:2 ↔ base_nivel2:1
- Mate:187: SoporteServo:2 ↔ base_nivel2:1
- Mate:188: SoporteServo:2 ↔ Tower Pro MG90S Micro servo:1
- Mate:189: ISO 4032 M2:14 ↔ ISO 4762 M2 x 8:2
- Mate:190: ISO 4032 M2:14 ↔ base_powerboost:1
- Mate:191: ISO 4032 M2:15 ↔ ISO 4762 M2 x 8:1
- Mate:192: ISO 4032 M2:15 ↔ base_powerboost:1
- Mate:193: ISO 4032 M2:16 ↔ ISO 4762 M2 x 12:3
- Mate:194: ISO 4032 M2:16 ↔ base_powerboost:1
- Mate:195: ISO 4032 M2:17 ↔ ISO 4762 M2 x 12:2
- Mate:196: ISO 4032 M2:17 ↔ base_powerboost:1
- Mate:197: ISO 4032 M2:16 ↔ powerboost:1
- Mate:199: ISO 4032 M3:17 ↔ base_chasis_v4-dimsAjustadas:1
- Mate:201: ISO 4032 M3:18 ↔ base_chasis_v4-dimsAjustadas:1
- Mate:202: ISO 4762 M3 x 8:1 ↔ cremallera-01:1
- Mate:203: ISO 4762 M3 x 8:1 ↔ sujetador_cremallera:1
- Mate:204: ISO 4762 M3 x 8:2 ↔ cremallera-01:1
- Mate:205: ISO 4762 M3 x 8:2 ↔ sujetador_cremallera:1
- Mate:206: ISO 4762 M3 x 8:1 ↔ ISO 4032 M3:11
- Mate:207: ISO 4762 M3 x 8:2 ↔ ISO 4032 M3:12
- Mate:208: SoporteServo:1 ↔ ISO 4032 M2:13
- Mate:209: SoporteServo:2 ↔ ISO 4032 M2:12
## Named parameters: Finish10_Area = 2.70707, Finish11_Area = 34.5669, Finish12_Area = 34.5669, Finish13_Area = 34.5669, Finish14_Area = 241.215, Finish15_Area = 241.215, Finish16_Area = 0.56205, Finish17_Area = 0.56205, Finish18_Area = 1.1241, Finish19_Area = 1.1241, Finish1_Area = 453.766, Finish20_Area = 5.43503, Finish21_Area = 5.43503, Finish2_Area = 0.953201, Finish2_Thickness = 0.05 mm, Finish3_Area = 2.8596, Finish3_Thickness = 0.05 mm, Finish4_Area = 412.295, Finish5_Area = 41.4714, Finish6_Area = 2.70707, Finish7_Area = 13.3512, Finish8_Area = 13.3512, Finish9_Area = 2.70707
note: some values were not read from the file. Shown as the stored number, unit unknown: "Finish10_Area", "Finish11_Area", "Finish12_Area", "Finish13_Area", "Finish14_Area", "Finish15_Area", "Finish16_Area", "Finish17_Area", "Finish18_Area", "Finish19_Area", "Finish1_Area", "Finish20_Area", "Finish21_Area", "Finish2_Area", "Finish3_Area", "Finish4_Area", "Finish5_Area", "Finish6_Area", "Finish7_Area", "Finish8_Area", "Finish9_Area".
